# Autodesk Inventor assembly: Skrzydło
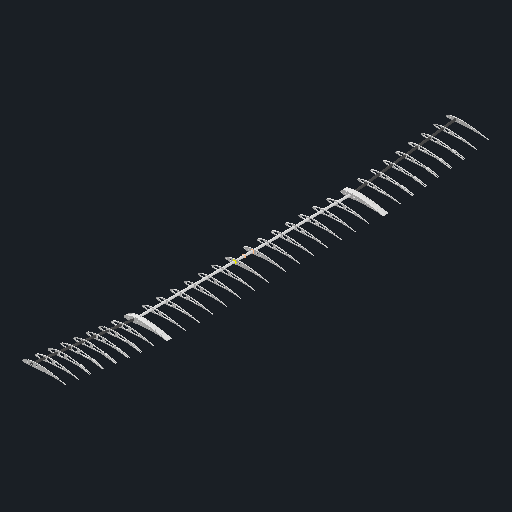
[picture p0: Inventor's stored thumbnail of the model, 512x512]
Saved by Autodesk Inventor 2023.2 (Build 272271030, 271C)
## iProperties
Created: 2023-01-05
Part Number: Skrzydło
Document SubType Name: Assembly
Designer: szykr
Author: szykr
## Documents named in this file (7)
- C:\Users\Maciej\Desktop\samolot\Solaris\Solaris\new model\Skrzydło.iam
- C:\Users\Maciej\Desktop\samolot\Solaris\Solaris\new model\wingspar.ipt
- C:\Users\Maciej\Desktop\samolot\Solaris\Solaris\new model\Żerbo montaż.ipt
- C:\Users\Maciej\Desktop\samolot\Solaris\Solaris\new model\Żebro default.ipt
- C:\Users\Maciej\Desktop\samolot\Solaris\Solaris\new model\kuplung.ipt
- C:\Users\Maciej\Desktop\samolot\Solaris\Solaris\new model\skrzydlo_ster.iam
- C:\Users\Maciej\Desktop\samolot\Solaris\Solaris\new model\Skrzydlo_ster_mir\skrzydlo_ster_MIR.iam
## Components (21 placed, 6 different names)
1. wingspar:1 — Insert:1, Insert:9, Insert:11, Insert:13
2. Żerbo montaż:1 — Insert:1, Insert:3, Insert:4
3. Żerbo montaż:3 — Insert:4
4. Żerbo montaż:5 — Insert:9, Insert:10
5. Żerbo montaż:6 — Insert:11, Insert:12
6. kuplung:1 — Insert:12, Insert:15
7. kuplung:2 — Insert:13, Insert:14
8. skrzydlo_ster:1 [sub-assembly] — Insert:14
9. skrzydlo_ster_MIR:1 [sub-assembly] — Insert:15
10. Żebro default:1 — Insert:3
11. Żebro default:2
12. Żebro default:3
13. Żebro default:4
14. Żebro default:5
15. Żebro default:6
16. Żebro default:7 — Insert:10
17. Żebro default:8
18. Żebro default:9
19. Żebro default:10
20. Żebro default:11
21. Żebro default:12
## Component patterns: (6 elements, first: Żebro default:1), (6 elements, first: Żebro default:7)
## Relationships (10: Insert 10)
- Insert:1 (-460 mm): wingspar:1 ↔ Żerbo montaż:1
- Insert:3 (-64.1429 mm): Żerbo montaż:1 ↔ Żebro default:1
- Insert:4 (449 mm): Żerbo montaż:1 ↔ Żerbo montaż:3
- Insert:9 (-460 mm): wingspar:1 ↔ Żerbo montaż:5
- Insert:10 (-64.1429 mm): Żerbo montaż:5 ↔ Żebro default:7
- Insert:11 (8 mm): wingspar:1 ↔ Żerbo montaż:6
- Insert:12: Żerbo montaż:6 ↔ kuplung:1
- Insert:13 (-8 mm): wingspar:1 ↔ kuplung:2
- Insert:14: kuplung:2 ↔ skrzydlo_ster:1
- Insert:15: kuplung:1 ↔ skrzydlo_ster_MIR:1
## Named parameters: ilosc_cala_zeber = 8, ilosc_zeber_pattern = 6, dlugosc_zeber = 449 mm, spacing = 64.14286 mm
